# Autodesk Inventor assembly: peg
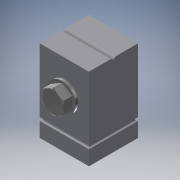
[picture p0: Inventor's stored thumbnail of the model, 180x180]
Saved by Autodesk Inventor 2019 (Build 230136000, 136)
## iProperties
Created: 2019-12-28
Part Number: peg
Material: Типовые
Document SubType Name: Assembly
Designer: stepa
Author: stepa
## Documents named in this file (3)
- C:\Users\stepa\Documents\Inventor\Shamisen\peg.iam
- C:\Users\stepa\Documents\Inventor\Shamisen\peg_half.ipt
- C:\Users\stepa\Documents\Inventor\Shamisen\peg\Мастер проектирования\Болтовое соединение1.iam
## Components (3 placed, 2 different names)
1. peg_half:1 — Совмещение:1, Заподлицо:1, Заподлицо:2
2. peg_half:2 — Совмещение:1, Заподлицо:1, Заподлицо:2, Совмещение:2, Совмещение:3
3. Болтовое соединение:1 [sub-assembly] — Совмещение:2, Совмещение:3
## Relationships (5: Mate 3, Flush 2)
- Совмещение:1 [Mate]: peg_half:1 ↔ peg_half:2
- Заподлицо:1 [Flush]: peg_half:1 ↔ peg_half:2
- Заподлицо:2 [Flush]: peg_half:1 ↔ peg_half:2
- Совмещение:2 [Mate]: peg_half:2 ↔ Болтовое соединение:1
- Совмещение:3 [Mate]: peg_half:2 ↔ Болтовое соединение:1
